# Autodesk Inventor assembly: Assembly1
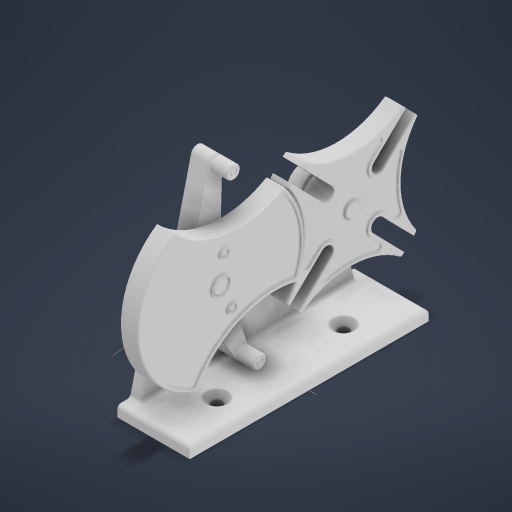
[picture p0: Inventor's stored thumbnail of the model, 512x512]
Saved by Autodesk Inventor 2023.2 (Build 272271000, 271)
## iProperties
Created: 2022-11-29
Part Number: Assembly1
Document SubType Name: Assembly
Designer: iusti
Author: iusti
## Documents named in this file (9)
- D:\Piese\Constantin Stancescu\018 Geneva drive\Assembly1.iam
- D:\Piese\Constantin Stancescu\018 Geneva drive\Support.ipt
- D:\Piese\Constantin Stancescu\018 Geneva drive\Malta cross.ipt
- D:\Piese\Constantin Stancescu\018 Geneva drive\Disk.ipt
- D:\Piese\Constantin Stancescu\018 Geneva drive\Lever.ipt
- D:\Piese\Constantin Stancescu\018 Geneva drive\Roller.ipt
- D:\Piese\Constantin Stancescu\018 Geneva drive\Pin.ipt
- D:\Piese\Constantin Stancescu\018 Geneva drive\Axle Small.ipt
- D:\Piese\Constantin Stancescu\018 Geneva drive\Axle Big.ipt
## Components (12 placed, 8 different names)
1. Support:1 — Insert:1, Insert:2, Insert:3, Insert:4
2. Malta cross:1 — Insert:4
3. Disk:1 — Insert:5, Insert:7, Insert:9
4. Lever:1 — Insert:3, Insert:5, Insert:6, Insert:8, Insert:10, Insert:11, Insert:12, Insert:13
5. Roller:1 — Insert:13
6. Roller:2 — Insert:12
7. Pin:1 — Insert:6, Insert:7
8. Pin:2 — Insert:8, Insert:9
9. Axle Small:1 — Insert:10
10. Axle Small:2 — Insert:11
11. Axle Big:1 — Insert:1
12. Axle Big:2 — Insert:2
## Relationships (13: Insert 13)
- Insert:1: Support:1 ↔ Axle Big:1
- Insert:2: Support:1 ↔ Axle Big:2
- Insert:3: Support:1 ↔ Lever:1
- Insert:4: Support:1 ↔ Malta cross:1
- Insert:5: Disk:1 ↔ Lever:1
- Insert:6: Lever:1 ↔ Pin:1
- Insert:7: Disk:1 ↔ Pin:1
- Insert:8: Lever:1 ↔ Pin:2
- Insert:9: Disk:1 ↔ Pin:2
- Insert:10: Lever:1 ↔ Axle Small:1
- Insert:11: Lever:1 ↔ Axle Small:2
- Insert:12: Lever:1 ↔ Roller:2
- Insert:13: Lever:1 ↔ Roller:1
